# Autodesk Inventor assembly: Assembly
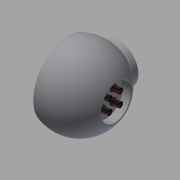
[picture p0: Inventor's stored thumbnail of the model, 180x180]
Saved by Autodesk Inventor 2020 (Build 240168000, 168)
## iProperties
Created: 2020-03-09
Part Number: Assembly
Document SubType Name: Assembly
Designer: user
Author: user
## Documents named in this file (5)
- D:\Documents\Github\Arduino-Smart-light\3DModel\Assembly.iam
- D:\Documents\Github\Arduino-Smart-light\3DModel\Lamp body.ipt
- C:\Users\user\Google Drive\Projects\3d\4 Projects\AA Done\.Parts\Potentiometer RK097N.ipt
- D:\Documents\Github\Arduino-Smart-light\3DModel\Lamp stand.ipt
- C:\Users\user\Google Drive\Projects\3d\4 Projects\AA Done\.Parts\Potentiometer cap.ipt
## Components (10 placed, 4 different names)
1. Lamp body:1 — Mate:8, Mate:9, Mate:16, Mate:21, Mate:22, Mate:23, Mate:24, Mate:25
2. Lamp stand:2 — Mate:8, Mate:11, Mate:12, Flush:3, Mate:21
3. Potentiometer RK097N:5 — Flush:1, Flush:2, Mate:9, Angle:1, Mate:23, Flush:8, Mate:28
4. Potentiometer RK097N:6 — Flush:2, Angle:1, Angle:2, Mate:25, Flush:8, Mate:29
5. Potentiometer RK097N:7 — Flush:1, Angle:2, Flush:7, Angle:4, Mate:22, Mate:27
6. Potentiometer RK097N:8 — Flush:7, Angle:4, Mate:24, Mate:26
7. Potentiometer cap:5 — Flush:4, Flush:6, Mate:29
8. Potentiometer cap:6 — Mate:16, Flush:4, Flush:5, Mate:27
9. Potentiometer cap:7 — Flush:5, Mate:28
10. Potentiometer cap:8 — Flush:6, Mate:26
## Relationships (25: Mate 14, Flush 8, Angle 3)
- Flush:1: Potentiometer RK097N:5 ↔ Potentiometer RK097N:7
- Flush:2: Potentiometer RK097N:5 ↔ Potentiometer RK097N:6
- Mate:8: Lamp body:1 ↔ Lamp stand:2
- Mate:9: Lamp body:1 ↔ Potentiometer RK097N:5
- Mate:11: Lamp stand:2
- Mate:12: Lamp stand:2
- Flush:3: Lamp stand:2
- Angle:1 (0 deg): Potentiometer RK097N:5 ↔ Potentiometer RK097N:6
- Angle:2 (0 deg): Potentiometer RK097N:6 ↔ Potentiometer RK097N:7
- Mate:16 (0.2 mm): Lamp body:1 ↔ Potentiometer cap:6
- Flush:4: Potentiometer cap:5 ↔ Potentiometer cap:6
- Flush:5: Potentiometer cap:6 ↔ Potentiometer cap:7
- Flush:6: Potentiometer cap:5 ↔ Potentiometer cap:8
- Flush:7: Potentiometer RK097N:7 ↔ Potentiometer RK097N:8
- Angle:4 (0 deg): Potentiometer RK097N:7 ↔ Potentiometer RK097N:8
- Mate:21: Lamp body:1 ↔ Lamp stand:2
- Mate:22: Lamp body:1 ↔ Potentiometer RK097N:7
- Mate:23: Lamp body:1 ↔ Potentiometer RK097N:5
- Mate:24: Lamp body:1 ↔ Potentiometer RK097N:8
- Mate:25: Lamp body:1 ↔ Potentiometer RK097N:6
- Flush:8: Potentiometer RK097N:5 ↔ Potentiometer RK097N:6
- Mate:26: Potentiometer RK097N:8 ↔ Potentiometer cap:8
- Mate:27: Potentiometer RK097N:7 ↔ Potentiometer cap:6
- Mate:28: Potentiometer RK097N:5 ↔ Potentiometer cap:7
- Mate:29: Potentiometer RK097N:6 ↔ Potentiometer cap:5
